# Autodesk Inventor assembly: Platform Assembly
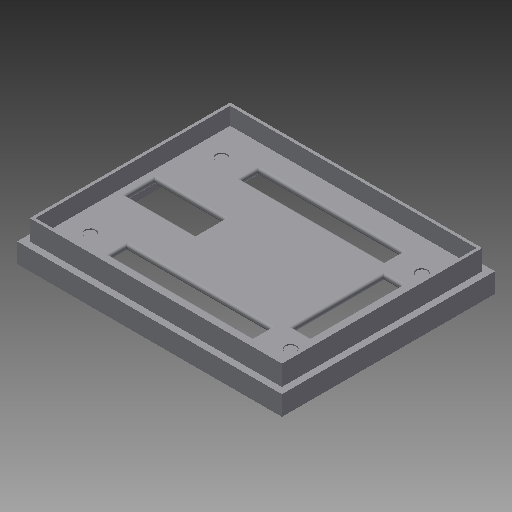
[picture p0: Inventor's stored thumbnail of the model, 512x512]
Saved by Autodesk Inventor 2017 (Build 210142000, 142)
## iProperties
Created: 2018-03-22
Part Number: Platform Assembly
Document SubType Name: Assembly
Designer: Arjuna
Author: Arjuna
## Documents named in this file (4)
- D:\Users\Arjuna\Documents\NTU\FYP\Hardware\Platform Assembly.iam
- D:\Users\Arjuna\Documents\NTU\FYP\Hardware\Platform-bottom.ipt
- D:\Users\Arjuna\Documents\NTU\FYP\Hardware\Platform-top.ipt
- D:\Users\Arjuna\Documents\NTU\FYP\Hardware\Platform Pin.ipt
## Components (6 placed, 3 different names)
1. Platform-bottom:1 — Mate:1, Flush:1, Flush:2, Flush:3, Insert:5, Insert:6
2. Platform-top:1 — Mate:1, Insert:1, Insert:2, Insert:3, Insert:4
3. Platform Pin:1 — Insert:1
4. Platform Pin:2 — Insert:2, Insert:6
5. Platform Pin:3 — Insert:3
6. Platform Pin:4 — Insert:4, Insert:5
## Relationships (10: Insert 6, Flush 3, Mate 1)
- Mate:1: Platform-bottom:1 ↔ Platform-top:1
- Insert:1: Platform-top:1 ↔ Platform Pin:1
- Insert:2: Platform-top:1 ↔ Platform Pin:2
- Insert:3: Platform-top:1 ↔ Platform Pin:3
- Insert:4: Platform-top:1 ↔ Platform Pin:4
- Flush:1: Platform-bottom:1
- Flush:2: Platform-bottom:1
- Flush:3: Platform-bottom:1
- Insert:5: Platform-bottom:1 ↔ Platform Pin:4
- Insert:6: Platform-bottom:1 ↔ Platform Pin:2
